# Autodesk Inventor assembly: wheel_molds_outer_rings_cut
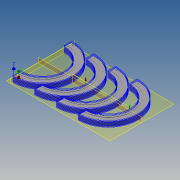
[picture p0: Inventor's stored thumbnail of the model, 180x180]
Saved by Autodesk Inventor 2014 SP2 (Build 180246200, 246)
## iProperties
Created: 2014-08-02
Part Number: wheel_molds_outer_rings_cut
Document SubType Name: Assembly
Designer: Yann
Author: Yann
## Documents named in this file (2)
- C:\Users\Yann\Documents\GitHub\PowerTrike_US\Workspaces\Espace de travail\Source\Front_train\wheel_molds_outer_rings_cut.iam
- C:\Users\Yann\Documents\GitHub\PowerTrike_US\Workspaces\Espace de travail\Source\Front_train\wheel_rim_mold_B_Prime.ipt
## Components (4 placed, 1 different names)
1. wheel_rim_mold_B_Prime:1 — Placage:4, Placage:5, Tangente:2, Tangente:3
2. wheel_rim_mold_B_Prime:2 — Placage:3, Placage:6, Tangente:3
3. wheel_rim_mold_B_Prime:3 — Placage:2, Placage:7, Tangente:1, Tangente:2
4. wheel_rim_mold_B_Prime:4 — Placage:1, Placage:8, Placage:9, Tangente:1
## Relationships (12: Mate 9, Tangent 3)
- Placage:1 [Mate]: wheel_rim_mold_B_Prime:4
- Placage:2 [Mate]: wheel_rim_mold_B_Prime:3
- Placage:3 [Mate]: wheel_rim_mold_B_Prime:2
- Placage:4 [Mate]: wheel_rim_mold_B_Prime:1
- Placage:5 [Mate]: wheel_rim_mold_B_Prime:1
- Placage:6 [Mate]: wheel_rim_mold_B_Prime:2
- Placage:7 [Mate]: wheel_rim_mold_B_Prime:3
- Placage:8 [Mate]: wheel_rim_mold_B_Prime:4
- Placage:9 [Mate]: wheel_rim_mold_B_Prime:4
- Tangente:1 (19.05 mm): wheel_rim_mold_B_Prime:3 ↔ wheel_rim_mold_B_Prime:4
- Tangente:2 (19.05 mm): wheel_rim_mold_B_Prime:1 ↔ wheel_rim_mold_B_Prime:3
- Tangente:3 (19.05 mm): wheel_rim_mold_B_Prime:1 ↔ wheel_rim_mold_B_Prime:2
